# Autodesk Inventor assembly: PumpConcept
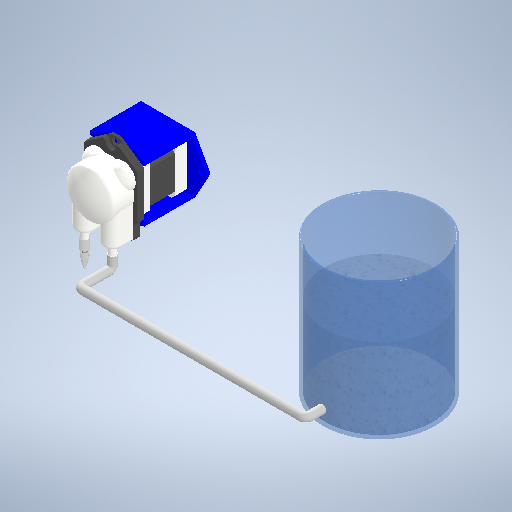
[picture p0: Inventor's stored thumbnail of the model, 512x512]
Saved by Autodesk Inventor 2025.2 (Build 292293000, 293)
## iProperties
Created: 2025-05-29
Part Number: PumpConcept
Document SubType Name: Assembly
Designer: Simon
Author: Simon
## Documents named in this file (8)
- C:\Users\Simon\OneDrive\Documents\Inventor\Skripsie2025\Extruder Concept 3\PumpConcept.iam
- C:\Users\Simon\OneDrive\Documents\Inventor\Skripsie2025\PartsFolder\Peristaltic Pump\Peristaltic Pump Assembly.iam
- C:\Users\Simon\OneDrive\Documents\Inventor\Skripsie2025\Extruder Concept 3\Gel.ipt
- C:\Users\Simon\OneDrive\Documents\Inventor\Skripsie2025\Extruder Concept 3\Reservoir.ipt
- C:\Users\Simon\OneDrive\Documents\Inventor\Skripsie2025\Extruder Concept 3\Pipe.ipt
- C:\Users\Simon\OneDrive\Documents\Inventor\Skripsie2025\Extruder Concept 3\Mount.ipt
- C:\Users\Simon\OneDrive\Documents\Inventor\Skripsie2025\Extruder Concept 3\Nozzle.ipt
- C:\Users\Simon\OneDrive\Documents\Inventor\Skripsie2025\Extruder Concept 3\NozzleAttachment.ipt
## Components (7 placed, 7 different names)
1. Peristaltic Pump Assembly:1 [sub-assembly] — Mate:1, Mate:2, Mate:3, Flush:1, Mate:7, Angle:1, Angle:3, Tangent:2, Mate:9, Mate:11, Mate:12, Mate:13, Mate:14, Flush:4, Angle:4
2. Gel:1 — Mate:4, Mate:5
3. Reservoir:1 — Mate:4, Mate:5, Mate:6, Tangent:1, Flush:2, Flush:3, Mate:10
4. Pipe:1 — Mate:9, Mate:10
5. Mount:1 — Mate:11, Mate:12, Mate:13
6. Nozzle:1 — Mate:15, Mate:16, Angle:4
7. NozzleAttachment:1 — Mate:14, Flush:4, Mate:15, Mate:16
## Relationships (26: Mate 16, Flush 4, Angle 4, Tangent 2)
- Mate:1: Peristaltic Pump Assembly:1
- Mate:2: Peristaltic Pump Assembly:1
- Mate:3: Peristaltic Pump Assembly:1
- Mate:4: Gel:1 ↔ Reservoir:1
- Mate:5: Gel:1 ↔ Reservoir:1
- Mate:6 (-40 mm): Reservoir:1
- Flush:1: Peristaltic Pump Assembly:1
- Mate:7: Peristaltic Pump Assembly:1
- Angle:1 (0 deg): Peristaltic Pump Assembly:1
- Angle:2 (0 deg)
- Tangent:1: Reservoir:1
- Mate:8 (200 mm)
- Angle:3 (0 deg): Peristaltic Pump Assembly:1
- Tangent:2: Peristaltic Pump Assembly:1
- Flush:2: Reservoir:1
- Flush:3: Reservoir:1
- Mate:9: Peristaltic Pump Assembly:1 ↔ Pipe:1
- Mate:10: Reservoir:1 ↔ Pipe:1
- Mate:11: Peristaltic Pump Assembly:1 ↔ Mount:1
- Mate:12: Peristaltic Pump Assembly:1 ↔ Mount:1
- Mate:13: Peristaltic Pump Assembly:1 ↔ Mount:1
- Mate:14: Peristaltic Pump Assembly:1 ↔ NozzleAttachment:1
- Flush:4 (-0.1 mm): Peristaltic Pump Assembly:1 ↔ NozzleAttachment:1
- Mate:15: Nozzle:1 ↔ NozzleAttachment:1
- Mate:16: Nozzle:1 ↔ NozzleAttachment:1
- Angle:4 (0 deg): Peristaltic Pump Assembly:1 ↔ Nozzle:1
